# Autodesk Inventor assembly: Марш-02
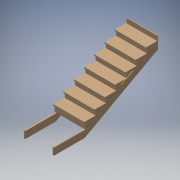
[picture p0: Inventor's stored thumbnail of the model, 180x180]
Saved by Autodesk Inventor 2019 (Build 230136000, 136)
## iProperties
Created: 2018-10-10
Part Number: Марш-02
Material: Типовые
Document SubType Name: Assembly
Designer: Андреев Н.Л.
Author: Андреев Н.Л.
## Documents named in this file (13)
- C:\Users\andrnl\Documents\Inventor\Мурзин\Марш.iam
- C:\Users\andrnl\Documents\Inventor\Мурзин\Проступь\Проступь-01.ipt
- C:\Users\andrnl\Documents\Inventor\Мурзин\Проступь.ipt
- C:\Users\andrnl\Documents\Inventor\Мурзин\Подступенок\Подступенок-01.ipt
- C:\Users\andrnl\Documents\Inventor\Мурзин\Подступенок.ipt
- C:\Users\andrnl\Documents\Inventor\Мурзин\Подступенок\Подступенок-02.ipt
- C:\Users\andrnl\Documents\Inventor\Мурзин\Косоур\Косоур-01.ipt
- C:\Users\andrnl\Documents\Inventor\Мурзин\Косоур.ipt
- C:\Users\andrnl\Documents\Inventor\Мурзин\Косоур\Косоур-02.ipt
- C:\Users\andrnl\Documents\Inventor\Мурзин\Подступенок\Подступенок-03.ipt
- Марш-01.iam
- Марш-02.iam
- C:\Users\andrnl\Documents\Inventor\Мурзин\Лестница Мурзин.xlsx
## Components (20 placed, 6 different names)
1. Подступенок-02:8 — Заподлицо:7, Заподлицо:8, Совмещение:8
2. Подступенок-03:10 — Заподлицо:12, Совмещение:14, Совмещение:15, Совмещение:17
3. Косоур-01:1 — Заподлицо:13, Совмещение:16, Совмещение:17, Заподлицо:15, Заподлицо:16
4. Косоур-01:2 — Заподлицо:14, Заподлицо:15, Заподлицо:16
5. Косоур-02:3 — Совмещение:18, Совмещение:19, Совмещение:20, Заподлицо:18, Заподлицо:19
6. Косоур-02:4 — Заподлицо:17, Заподлицо:18, Заподлицо:19
7. Проступь-01:1 — Заподлицо:1, Заподлицо:2, Заподлицо:3, Заподлицо:5, Совмещение:1, Совмещение:13, Совмещение:7, Совмещение:8, Заподлицо:11, Совмещение:9, Совмещение:14, Совмещение:15, Совмещение:16, Заподлицо:14, Совмещение:20, Заподлицо:17
8. Проступь-01:2
9. Проступь-01:3
10. Проступь-01:4
11. Проступь-01:5
12. Проступь-01:6
13. Проступь-01:7
14. Подступенок-01:1 — Заподлицо:10, Совмещение:13, Совмещение:7, Совмещение:19
15. Подступенок-01:2
16. Подступенок-01:3
17. Подступенок-01:4
18. Подступенок-01:5
19. Подступенок-01:6
20. Подступенок-01:7
## Component patterns: (7 elements, first: Проступь-01:1), (7 elements, first: Подступенок-01:1)
## Relationships (31: Flush 16, Mate 15)
- Заподлицо:1 [Flush]: Проступь-01:1
- Заподлицо:2 [Flush]: Проступь-01:1
- Заподлицо:3 [Flush] (-3087.5 mm): Проступь-01:1
- Заподлицо:5 [Flush] (-296.8 mm): Проступь-01:1
- Совмещение:1 [Mate]: Проступь-01:1
- Совмещение:2 [Mate]
- Совмещение:3 [Mate]
- Заподлицо:10 [Flush]: Подступенок-01:1
- Совмещение:13 [Mate]: Проступь-01:1 ↔ Подступенок-01:1
- Совмещение:7 [Mate]: Проступь-01:1 ↔ Подступенок-01:1
- Заподлицо:7 [Flush]: Подступенок-02:8
- Заподлицо:8 [Flush]: Подступенок-02:8
- Совмещение:8 [Mate] (-3264.8 mm): Подступенок-02:8 ↔ Проступь-01:1
- Заподлицо:11 [Flush] (-162.5 mm): Проступь-01:1
- Совмещение:9 [Mate]: Проступь-01:1
- Совмещение:10 [Mate]
- Заподлицо:12 [Flush]: Подступенок-03:10
- Совмещение:14 [Mate]: Подступенок-03:10 ↔ Проступь-01:1
- Совмещение:15 [Mate] (-162.5 mm): Подступенок-03:10 ↔ Проступь-01:1
- Заподлицо:13 [Flush]: Косоур-01:1
- Совмещение:16 [Mate]: Косоур-01:1 ↔ Проступь-01:1
- Совмещение:17 [Mate]: Подступенок-03:10 ↔ Косоур-01:1
- Заподлицо:14 [Flush] (30 mm): Косоур-01:2 ↔ Проступь-01:1
- Заподлицо:15 [Flush]: Косоур-01:1 ↔ Косоур-01:2
- Заподлицо:16 [Flush]: Косоур-01:1 ↔ Косоур-01:2
- Совмещение:18 [Mate]: Косоур-02:3
- Совмещение:19 [Mate]: Косоур-02:3 ↔ Подступенок-01:1
- Совмещение:20 [Mate]: Косоур-02:3 ↔ Проступь-01:1
- Заподлицо:17 [Flush] (30 mm): Косоур-02:4 ↔ Проступь-01:1
- Заподлицо:18 [Flush]: Косоур-02:3 ↔ Косоур-02:4
- Заподлицо:19 [Flush]: Косоур-02:3 ↔ Косоур-02:4
## Named parameters: Уровень = -3087.5 mm, зУр2Эт = 3250 mm, зДл = 3000 mm, зШир = 2000 mm, пДлПроступи = 900 mm, пПодъемов = 20, пПодъем = 162.5 mm, пХод = 296.8 mm, пЭффШаг = 621.8 mm, пСвес = 30.2 mm, пТолПроступи = 40 mm, пТолКосоура = 40 mm, пТолСтолба = 90 mm, пТолБалясины = 40 mm, пШирКосоура = 300 mm, пОтступСтен = 5 mm, пДиаг = 338.3733 mm, пПлощадка = 1, пПодъемов2 = 7, пВыход2Ур = 1, пПодъемов1 = 11, пШирПроступи = 327 mm, пТолПодступенка = 17.4 mm, пШипПодступ = 10 mm, пОтступШипа = 50 mm, пГлубПаза = 12 mm, пОтступПодступ = 10 mm, пОтступОтСтен = 5 mm, пДлПлощадки = 1990 mm, Проступей = 7, Подступенков = 7, пТолПричала = 17.4 mm, зТолПерекрытия = 300 mm, пСвесВбок = 30 mm
